# Autodesk Inventor assembly: Carte Capteurs
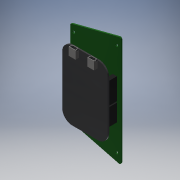
[picture p0: Inventor's stored thumbnail of the model, 180x180]
Saved by Autodesk Inventor 2019 (Build 230136000, 136)
## iProperties
Created: 2019-08-29
Part Number: Carte Capteurs
Material: Générique
Document SubType Name: Assembly
Designer: Sébastien DI MERCURIO
Author: Sébastien DI MERCURIO
## Documents named in this file (3)
- D:\Users\dimercur\Documents locaux\Travail\git\insa-nxpcup-1\meca\Inventor\Carte Capteurs.iam
- D:\Users\dimercur\Documents locaux\Travail\git\insa-nxpcup-1\pcb\Carte_Capteurs\Carte_Capteurs.ipt
- D:\Users\dimercur\Documents locaux\Travail\git\insa-nxpcup-1\meca\Inventor\FRDM-KL25Z.ipt
## Components (2 placed, 2 different names)
1. Carte_Capteurs:1 — Placage:1, Angle:1, Angle:2, Placage:2, Placage:3
2. FRDM-KL25Z:1 — Placage:1, Angle:1, Placage:2, Placage:3
## Relationships (5: Mate 3, Angle 2)
- Placage:1 [Mate]: Carte_Capteurs:1 ↔ FRDM-KL25Z:1
- Angle:1 (0 deg): Carte_Capteurs:1 ↔ FRDM-KL25Z:1
- Angle:2 (90 deg): Carte_Capteurs:1
- Placage:2 [Mate] (5.76 mm): Carte_Capteurs:1 ↔ FRDM-KL25Z:1
- Placage:3 [Mate] (29.74 mm): Carte_Capteurs:1 ↔ FRDM-KL25Z:1
